# Autodesk Inventor assembly: Assembly7
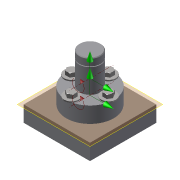
[picture p0: Inventor's stored thumbnail of the model, 180x180]
Saved by Autodesk Inventor 2017 (Build 210142000, 142)
## iProperties
Created: 2016-07-28
Part Number: Assembly7
Document SubType Name: Assembly
Designer: Tutorial Books
Author: Tutorial Books
## Documents named in this file (5)
- C:\Users\anand\Documents\Inventor\Autodesk Inventor 2017 Learn by doing\C07_tut1\Assembly7.iam
- C:\Users\anand\Documents\Inventor\Autodesk Inventor 2017 Learn by doing\C07_tut1\Base.ipt
- C:\Users\anand\Documents\Inventor\Autodesk Inventor 2017 Learn by doing\C07_tut1\Spacer.ipt
- C:\Users\anand\Documents\Inventor\Autodesk Inventor 2017 Learn by doing\C07_tut1\Shoulder Screw.ipt
- C:\Users\anand\Documents\Inventor\Autodesk Inventor 2017 Learn by doing\C07_tut1\Assembly7\Design Accelerator\Bolted Connection1.iam
## Components (7 placed, 4 different names)
1. Base:1 — Flush:1, Flush:4, Mate:4, Mate:5, Mate:6
2. Spacer:1 — Mate:5, Mate:6, Flush:6
3. Shoulder Screw:1 — Flush:4, Mate:4, Flush:5
4. Bolted Connection:1 [sub-assembly]
5. Bolted Connection:2 [sub-assembly]
6. Bolted Connection:3 [sub-assembly]
7. Bolted Connection:4 [sub-assembly]
## Component patterns: (4 elements, first: Bolted Connection:1)
## Relationships (7: Flush 4, Mate 3)
- Flush:1: Base:1
- Flush:4: Base:1 ↔ Shoulder Screw:1
- Mate:4: Base:1 ↔ Shoulder Screw:1
- Flush:5: Shoulder Screw:1
- Mate:5: Base:1 ↔ Spacer:1
- Mate:6: Base:1 ↔ Spacer:1
- Flush:6: Spacer:1
